# Autodesk Inventor assembly: Assembly2
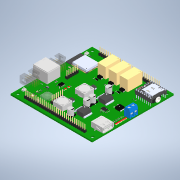
[picture p0: Inventor's stored thumbnail of the model, 180x180]
Saved by Autodesk Inventor 2021 (Build 250183000, 183)
## iProperties
Created: 2023-08-06
Part Number: Assembly2
Document SubType Name: Assembly
Designer: michal
Author: michal
## Documents named in this file (3)
- C:\Users\micha\OneDrive\Dokumenty\GitHub\escape_room_hw_v2\Enclosure\Commercial\Assembly2.iam
- C:\Users\micha\Downloads\ESP32-RGBW-WS2812b-LED-controller-main\main_board.iam
- C:\Users\micha\AppData\Local\Temp\Rar$DIa0.840\2-338556-1.ipt
## Components (2 placed, 2 different names)
1. main_board:1 [sub-assembly] — Mate:1, Flush:1
2. 2-338556-1:1 — Mate:1, Flush:1
## Relationships (2: Mate 1, Flush 1)
- Mate:1: main_board:1 ↔ 2-338556-1:1
- Flush:1 (-0.54 mm): main_board:1 ↔ 2-338556-1:1
